# Autodesk Inventor assembly: панель_электроники
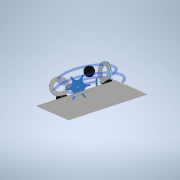
[picture p0: Inventor's stored thumbnail of the model, 180x180]
Saved by Autodesk Inventor 2021.1 (Build 251245010, 245A)
## iProperties
Created: 2022-11-16
Part Number: панель_электроники
Document SubType Name: Assembly
Designer: zmoze
Author: zmoze
## Documents named in this file (7)
- C:\Users\zmoze\OneDrive\Рабочий стол\GrabCAD\Smile_2022-2023\панель_электроники.iam
- C:\Users\zmoze\OneDrive\Рабочий стол\GrabCAD\Smile_2022-2023\панель_электроники_и не только.ipt
- C:\Users\zmoze\OneDrive\Рабочий стол\GrabCAD\Smile_2022-2023\шаговый_мотор.ipt
- C:\Users\zmoze\OneDrive\Рабочий стол\GrabCAD\Smile_2022-2023\шестеренка_для_мозговорота.ipt
- C:\Users\zmoze\OneDrive\Рабочий стол\GrabCAD\Smile_2022-2023\держалка_мозговорота.iam
- C:\Users\zmoze\OneDrive\Рабочий стол\GrabCAD\Smile_2022-2023\трубочки_мозговорота.ipt
- C:\Users\zmoze\OneDrive\Рабочий стол\GrabCAD\Smile_2022-2023\мячик_для_тенниса.ipt
## Components (8 placed, 6 different names)
1. панель_электроники_и не только:1 — Совмещение:5, Совмещение:6, Совмещение:7, Совмещение:8, Совмещение:12, Совмещение:13, Совмещение:14
2. шаговый_мотор:1 — Совмещение:1, Совмещение:2, Совмещение:5, Совмещение:12
3. шестеренка_для_мозговорота:1 — Совмещение:1, Совмещение:2, Совмещение:13
4. трубочки_мозговорота:1 — Совмещение:14
5. мячик_для_тенниса:1
6. держалка_мозговорота:1 [sub-assembly] — Совмещение:6, Совмещение:7, Совмещение:8
7. держалка_мозговорота:2 [sub-assembly]
8. держалка_мозговорота:3 [sub-assembly]
## Component patterns: (3 elements, first: держалка_мозговорота:1)
## Relationships (9: Mate 9)
- Совмещение:1 [Mate]: шаговый_мотор:1 ↔ шестеренка_для_мозговорота:1
- Совмещение:2 [Mate]: шаговый_мотор:1 ↔ шестеренка_для_мозговорота:1
- Совмещение:5 [Mate]: панель_электроники_и не только:1 ↔ шаговый_мотор:1
- Совмещение:6 [Mate]: панель_электроники_и не только:1 ↔ держалка_мозговорота:1
- Совмещение:7 [Mate]: панель_электроники_и не только:1 ↔ держалка_мозговорота:1
- Совмещение:8 [Mate] (100 mm): панель_электроники_и не только:1 ↔ держалка_мозговорота:1
- Совмещение:12 [Mate]: панель_электроники_и не только:1 ↔ шаговый_мотор:1
- Совмещение:13 [Mate] (-100 mm): панель_электроники_и не только:1 ↔ шестеренка_для_мозговорота:1
- Совмещение:14 [Mate]: панель_электроники_и не только:1 ↔ трубочки_мозговорота:1
